# Autodesk Inventor assembly: A2017_T4_02
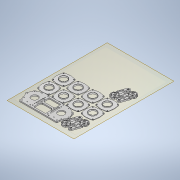
[picture p0: Inventor's stored thumbnail of the model, 180x180]
Saved by Autodesk Inventor 2020 (Build 240168000, 168)
## iProperties
Created: 2021-08-27
Part Number: A2017_T4_02
Document SubType Name: Assembly
Designer: Masato
Author: Masato
## Documents named in this file (5)
- C:\Users\naoki\Documents\Inventor\CitBrains\git_clone\OpenPlatform4_0\付け根ロール_サブフレーム_1_3追加\OpenPlatform_ver3_0\cam\A2017_T4_02.iam
- C:\Users\naoki\Documents\Inventor\CitBrains\git_clone\OpenPlatform4_0\A2017_T4_02\OpenPlatform_ver3_0\cam\Disposable_Board.ipt
- C:\Users\naoki\Documents\Inventor\CitBrains\git_clone\OpenPlatform4_0\A2017_T4_02\OpenPlatform_ver3_0\LowerBody\Ankle\Ankle_side_pitch_frame.ipt
- C:\Users\naoki\Documents\Inventor\CitBrains\git_clone\OpenPlatform4_0\A2017_T4_02\OpenPlatform_ver3_0\UpperBody\Trunk\Trunk_lower_waisit_frame.ipt
- C:\Users\naoki\Documents\Inventor\CitBrains\git_clone\OpenPlatform4_0\A2017_T4_02\OpenPlatform_ver3_0\cam\付け根ロール_サブフレーム_1_3.ipt
## Components (14 placed, 4 different names)
1. Disposable_Board:1 — メイト:2, メイト:1, フラッシュ:1, フラッシュ:2, メイト:4, メイト:5, メイト:6, フラッシュ:3, 正接:1, 正接:2, 正接:3, 角度:1, メイト:8, 正接:5
2. Trunk_lower_waisit_frame:1 — メイト:4, フラッシュ:3, 正接:1, 正接:4, 正接:6
3. Ankle_side_pitch_frame:2 — メイト:5, メイト:7, 正接:2, 正接:4, 角度:1
4. Ankle_side_pitch_frame:1 — メイト:6, メイト:7, 正接:3
5. Ankle_side_pitch_frame:3
6. Ankle_side_pitch_frame:4
7. 付け根ロール_サブフレーム_1_3:1 — メイト:8, 正接:5, 正接:6, 角度:2
8. 付け根ロール_サブフレーム_1_3:2
9. 付け根ロール_サブフレーム_1_3:3
10. 付け根ロール_サブフレーム_1_3:4
11. 付け根ロール_サブフレーム_1_3:5
12. 付け根ロール_サブフレーム_1_3:6
13. 付け根ロール_サブフレーム_1_3:7
14. 付け根ロール_サブフレーム_1_3:8
## Component patterns: (2 elements, first: Ankle_side_pitch_frame:2 + Ankle_side_pitch_frame:1), (8 elements, first: 付け根ロール_サブフレーム_1_3:1)
## Relationships (18: Mate 7, Tangent 6, Flush 3, Angle 2)
- メイト:2 [Mate]: Disposable_Board:1
- メイト:1 [Mate]: Disposable_Board:1
- フラッシュ:1 [Flush]: Disposable_Board:1
- フラッシュ:2 [Flush]: Disposable_Board:1
- メイト:4 [Mate]: Disposable_Board:1 ↔ Trunk_lower_waisit_frame:1
- メイト:5 [Mate]: Disposable_Board:1 ↔ Ankle_side_pitch_frame:2
- メイト:6 [Mate]: Disposable_Board:1 ↔ Ankle_side_pitch_frame:1
- フラッシュ:3 [Flush] (2 mm): Disposable_Board:1 ↔ Trunk_lower_waisit_frame:1
- 正接:1 [Tangent] (2 mm): Disposable_Board:1 ↔ Trunk_lower_waisit_frame:1
- メイト:7 [Mate] (2.5 mm): Ankle_side_pitch_frame:2 ↔ Ankle_side_pitch_frame:1
- 正接:2 [Tangent] (2 mm): Disposable_Board:1 ↔ Ankle_side_pitch_frame:2
- 正接:3 [Tangent] (2 mm): Disposable_Board:1 ↔ Ankle_side_pitch_frame:1
- 正接:4 [Tangent] (2.5 mm): Trunk_lower_waisit_frame:1 ↔ Ankle_side_pitch_frame:2
- 角度:1 [Angle] (0 deg): Disposable_Board:1 ↔ Ankle_side_pitch_frame:2
- メイト:8 [Mate]: Disposable_Board:1 ↔ 付け根ロール_サブフレーム_1_3:1
- 正接:5 [Tangent] (2 mm): Disposable_Board:1 ↔ 付け根ロール_サブフレーム_1_3:1
- 正接:6 [Tangent] (2.5 mm): Trunk_lower_waisit_frame:1 ↔ 付け根ロール_サブフレーム_1_3:1
- 角度:2 [Angle] (45 deg): 付け根ロール_サブフレーム_1_3:1
